# Autodesk Inventor assembly: Assembly1
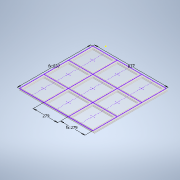
[picture p0: Inventor's stored thumbnail of the model, 180x180]
Saved by Autodesk Inventor 2021 (Build 250183000, 183)
## iProperties
Created: 2020-11-08
Part Number: Assembly1
Document SubType Name: Assembly
Designer: Wes
_SolveAssemblyDoc: Frame Generator Solve Assembly
_Version: 25.0.0
Author: Wes
## Documents named in this file (4)
- C:\Users\Wes\Documents\8020 DDR Pad\Assembly1.iam
- C:\Users\Wes\Documents\8020 DDR Pad\Part1.ipt
- C:\Users\Wes\Documents\8020 DDR Pad\Assembly1\Frame\Frame 1604978528816.iam
- C:\Users\Wes\Documents\8020 DDR Pad\Arrow Panel.ipt
## Components (11 placed, 3 different names)
1. Frame Sketch — Planar:1, Planar:2, Planar:3, Planar:4, Planar:5, Planar:6, Planar:7, Planar:8, Planar:9
2. 20mm Frame [sub-assembly]
3. Arrow Panel:1 — Planar:4
4. Arrow Panel:2 — Planar:8
5. Arrow Panel:3 — Planar:6
6. Arrow Panel:4 — Planar:1
7. Arrow Panel:5 — Planar:2
8. Arrow Panel:6 — Planar:5
9. Arrow Panel:7 — Planar:7
10. Arrow Panel:8 — Planar:3
11. Arrow Panel:9 — Planar:9
## Relationships (9: PlanarJoint 9)
- Planar:1: Frame Sketch ↔ Arrow Panel:4
- Planar:2: Frame Sketch ↔ Arrow Panel:5
- Planar:3: Frame Sketch ↔ Arrow Panel:8
- Planar:4: Frame Sketch ↔ Arrow Panel:1
- Planar:5: Frame Sketch ↔ Arrow Panel:6
- Planar:6: Frame Sketch ↔ Arrow Panel:3
- Planar:7: Frame Sketch ↔ Arrow Panel:7
- Planar:8: Frame Sketch ↔ Arrow Panel:2
- Planar:9: Frame Sketch ↔ Arrow Panel:9
